# Autodesk Inventor assembly: manipulator_asembly
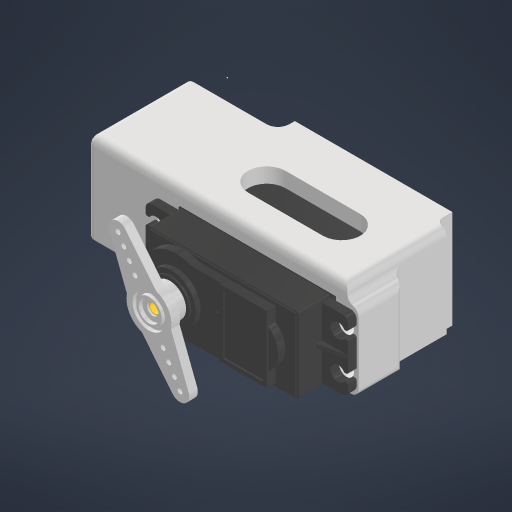
[picture p0: Inventor's stored thumbnail of the model, 512x512]
Saved by Autodesk Inventor 2024 (Build 280153000, 153)
## iProperties
Created: 2023-05-17
Part Number: manipulator_asembly
Document SubType Name: Assembly
Designer: user
Author: user
## Documents named in this file (3)
- D:\Docs\Robot\3d\manipulator\manipulator_asembly.iam
- D:\Docs\Robot\3d\manipulator\manipulator_asembly\manipulator_holder.ipt
- D:\Docs\Robot\3d\electronics\servo\MG996R SBORKA.iam
## Components (2 placed, 2 different names)
1. manipulator_holder:1 — Заподлицо:1, Заподлицо:2, Совмещение:1, Совмещение:3, Совмещение:4, Совмещение:5
2. MG996R SBORKA:1 [sub-assembly] — Совмещение:3, Совмещение:4, Совмещение:5
## Relationships (6: Mate 4, Flush 2)
- Заподлицо:1 [Flush]: manipulator_holder:1
- Заподлицо:2 [Flush]: manipulator_holder:1
- Совмещение:1 [Mate]: manipulator_holder:1
- Совмещение:3 [Mate]: manipulator_holder:1 ↔ MG996R SBORKA:1
- Совмещение:4 [Mate]: manipulator_holder:1 ↔ MG996R SBORKA:1
- Совмещение:5 [Mate]: manipulator_holder:1 ↔ MG996R SBORKA:1
